# Autodesk Inventor assembly: 初段_多段ギア
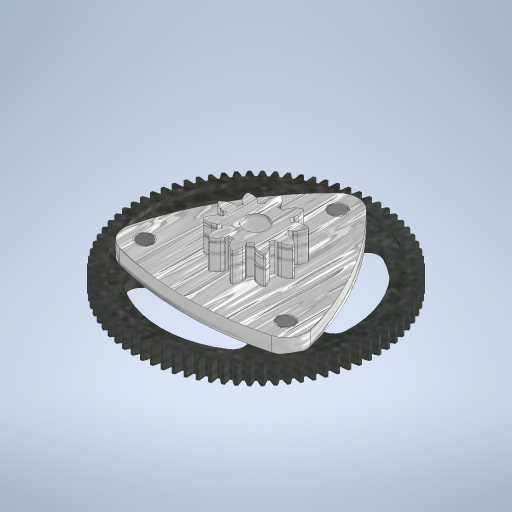
[picture p0: Inventor's stored thumbnail of the model, 512x512]
Saved by Autodesk Inventor 2023 (Build 270158030, 158C)
## iProperties
Created: 2022-01-11
Part Number: 初段_多段ギア
Document SubType Name: Assembly
Designer: acps
Mass: 16.1743 g
Surface Area: 43.5044 cm^2
Volume: 3.51662 cm^3
Density: 4.59937 g/cm^3
Author: acps
## Documents named in this file (4)
- C:\Users\muzho\Documents\srdc\srdc_2\アーム\ギア\初段_多段ギア.iam
- C:\Users\muzho\Documents\srdc\srdc_2\アーム\ギア\初段ギアm0.5z80.ipt
- C:\Users\muzho\Documents\srdc\srdc_2\アーム\ギア\m1z10t8.ipt
- C:\Users\muzho\Documents\srdc\srdc_2\ねじ\M3L4　超極低頭.ipt
## Components (5 placed, 3 different names)
1. 初段ギアm0.5z80:1 — メイト:1, 挿入:2, 挿入:3, 挿入:4, 挿入:5, 挿入:6
2. m1z10t8:1 — メイト:1, 挿入:3, 挿入:4
3. M3L4　超極低頭:1 — 挿入:6
4. M3L4　超極低頭:2 — 挿入:5
5. M3L4　超極低頭:3 — 挿入:2
## Relationships (6: Insert 5, Mate 1)
- メイト:1 [Mate]: 初段ギアm0.5z80:1 ↔ m1z10t8:1
- 挿入:2 [Insert]: 初段ギアm0.5z80:1 ↔ M3L4　超極低頭:3
- 挿入:3 [Insert]: 初段ギアm0.5z80:1 ↔ m1z10t8:1
- 挿入:4 [Insert]: 初段ギアm0.5z80:1 ↔ m1z10t8:1
- 挿入:5 [Insert]: 初段ギアm0.5z80:1 ↔ M3L4　超極低頭:2
- 挿入:6 [Insert]: 初段ギアm0.5z80:1 ↔ M3L4　超極低頭:1
